# Autodesk Inventor assembly: Gearbox Assembly
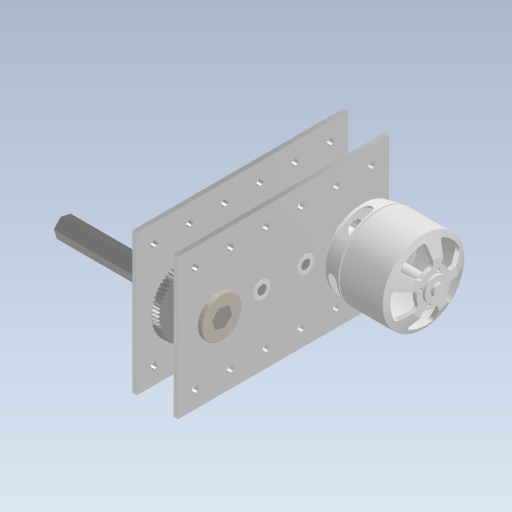
[picture p0: Inventor's stored thumbnail of the model, 512x512]
Saved by Autodesk Inventor 2023 (Build 270158000, 158)
## iProperties
Created: 2023-02-14
Part Number: Gearbox Assembly
Document SubType Name: Assembly
Designer: Dave
Mass: 682.162 g
Surface Area: 1267.39 cm^2
Volume: 183.282 cm^3
Density: 3.72192 g/cm^3
Author: Dave
## Documents named in this file (12)
- C:\Users\Dave\Documents\GitHub\BehrendURCMechanical\CAD\Chassis\GearBox\Final Gears and Assemblies\Gearbox Assembly.iam
- C:\Users\Dave\Documents\GitHub\BehrendURCMechanical\CAD\Chassis\GearBox\Final Gears and Assemblies\CH-1-01-20T_Drive Gear.ipt
- C:\Users\Dave\Documents\GitHub\BehrendURCMechanical\CAD\Chassis\GearBox\Final Gears and Assemblies\CH-1-01-60T_Output.ipt
- C:\Users\Dave\Documents\GitHub\BehrendURCMechanical\CAD\Chassis\GearBox\Final Gears and Assemblies\CH-1-01-20T_Idler.ipt
- C:\Users\Dave\Documents\GitHub\BehrendURCMechanical\CAD\Chassis\GearBox\Final Gears and Assemblies\CH-1-01-60T_Idler.ipt
- C:\Users\Dave\Documents\GitHub\BehrendURCMechanical\CAD\Chassis\GearBox\Housing\CH-1-02-RearGearboxHousingMotorSide.ipt
- C:\Users\Dave\Documents\GitHub\BehrendURCMechanical\CAD\Chassis\GearBox\Drive Motor Shaft Coupler.ipt
- C:\Users\Dave\Documents\GitHub\BehrendURCMechanical\CAD\Chassis\GearBox\Drive Motor.ipt
- C:\Users\Dave\Documents\GitHub\BehrendURCMechanical\CAD\Chassis\GearBox\Ch-1-01-0.5x4.5HexShaft.ipt
- C:\Users\Dave\Documents\GitHub\BehrendURCMechanical\CAD\Chassis\GearBox\CH-1-01-0.25x1.875SmoothShaft.ipt
- C:\Users\Dave\Documents\GitHub\BehrendURCMechanical\CAD\Chassis\GearBox\CH-1-01-0.5HexBearing.ipt
- C:\Users\Dave\Documents\GitHub\BehrendURCMechanical\CAD\Chassis\GearBox\CH-1-01-0.25IDSmoothBoreBearing.ipt
## Components (19 placed, 11 different names)
1. CH-1-01-20T_Drive Gear:1 — Insert:3
2. CH-1-01-60T_Output:1 — Mate:5, Mate:6, Mate:7
3. CH-1-01-20T_Idler:1 — Insert:1, Mate:2
4. CH-1-01-60T_Idler:1 — Insert:2, Mate:3, Mate:5
5. CH-1-01-20T_Idler:2 — Insert:2, Mate:4
6. CH-1-01-60T_Idler:2 — Insert:1, Mate:1, Mate:3
7. CH-1-02-RearGearboxHousingMotorSide:1 — Angle:1, Flush:1, Flush:2, Mate:2, Mate:4, Insert:5, Insert:6, Insert:7, Insert:10
8. CH-1-02-RearGearboxHousingMotorSide:2 — Flush:1, Flush:2, Mate:6, Mate:7, Insert:8, Insert:9, Insert:11
9. Drive Motor Shaft Coupler:1 — Insert:3, Insert:4, Mate:1, Insert:5
10. Drive Motor:1 — Insert:4
11. Ch-1-01-0.5x4.5HexShaft:1 — Flush:3, Mate:8, Mate:9
12. CH-1-01-0.25x1.875SmoothShaft:1 — Insert:13
13. CH-1-01-0.25x1.875SmoothShaft:2 — Insert:12
14. CH-1-01-0.5HexBearing:1 — Insert:11
15. CH-1-01-0.5HexBearing:2 — Insert:10, Flush:3, Mate:8, Mate:9
16. CH-1-01-0.25IDSmoothBoreBearing:1 — Insert:6, Insert:12
17. CH-1-01-0.25IDSmoothBoreBearing:2 — Insert:7, Insert:13
18. CH-1-01-0.25IDSmoothBoreBearing:3 — Insert:8
19. CH-1-01-0.25IDSmoothBoreBearing:4 — Insert:9
## Relationships (26: Insert 13, Mate 9, Flush 3, Angle 1)
- Insert:1: CH-1-01-20T_Idler:1 ↔ CH-1-01-60T_Idler:2
- Insert:2: CH-1-01-60T_Idler:1 ↔ CH-1-01-20T_Idler:2
- Insert:3: CH-1-01-20T_Drive Gear:1 ↔ Drive Motor Shaft Coupler:1
- Insert:4: Drive Motor Shaft Coupler:1 ↔ Drive Motor:1
- Angle:1 (0 deg): CH-1-02-RearGearboxHousingMotorSide:1
- Flush:1: CH-1-02-RearGearboxHousingMotorSide:1 ↔ CH-1-02-RearGearboxHousingMotorSide:2
- Flush:2: CH-1-02-RearGearboxHousingMotorSide:1 ↔ CH-1-02-RearGearboxHousingMotorSide:2
- Mate:1: CH-1-01-60T_Idler:2 ↔ Drive Motor Shaft Coupler:1
- Mate:2: CH-1-01-20T_Idler:1 ↔ CH-1-02-RearGearboxHousingMotorSide:1
- Mate:3: CH-1-01-60T_Idler:1 ↔ CH-1-01-60T_Idler:2
- Mate:4: CH-1-01-20T_Idler:2 ↔ CH-1-02-RearGearboxHousingMotorSide:1
- Mate:5: CH-1-01-60T_Output:1 ↔ CH-1-01-60T_Idler:1
- Mate:6: CH-1-01-60T_Output:1 ↔ CH-1-02-RearGearboxHousingMotorSide:2
- Mate:7 (1.5875 mm): CH-1-01-60T_Output:1 ↔ CH-1-02-RearGearboxHousingMotorSide:2
- Insert:5: CH-1-02-RearGearboxHousingMotorSide:1 ↔ Drive Motor Shaft Coupler:1
- Insert:6: CH-1-02-RearGearboxHousingMotorSide:1 ↔ CH-1-01-0.25IDSmoothBoreBearing:1
- Insert:7: CH-1-02-RearGearboxHousingMotorSide:1 ↔ CH-1-01-0.25IDSmoothBoreBearing:2
- Insert:8: CH-1-02-RearGearboxHousingMotorSide:2 ↔ CH-1-01-0.25IDSmoothBoreBearing:3
- Insert:9: CH-1-02-RearGearboxHousingMotorSide:2 ↔ CH-1-01-0.25IDSmoothBoreBearing:4
- Insert:10: CH-1-02-RearGearboxHousingMotorSide:1 ↔ CH-1-01-0.5HexBearing:2
- Insert:11: CH-1-02-RearGearboxHousingMotorSide:2 ↔ CH-1-01-0.5HexBearing:1
- Flush:3: Ch-1-01-0.5x4.5HexShaft:1 ↔ CH-1-01-0.5HexBearing:2
- Mate:8: Ch-1-01-0.5x4.5HexShaft:1 ↔ CH-1-01-0.5HexBearing:2
- Mate:9: Ch-1-01-0.5x4.5HexShaft:1 ↔ CH-1-01-0.5HexBearing:2
- Insert:12: CH-1-01-0.25x1.875SmoothShaft:2 ↔ CH-1-01-0.25IDSmoothBoreBearing:1
- Insert:13: CH-1-01-0.25x1.875SmoothShaft:1 ↔ CH-1-01-0.25IDSmoothBoreBearing:2
